# Autodesk Inventor assembly: WANYOIKE
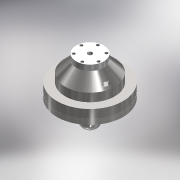
[picture p0: Inventor's stored thumbnail of the model, 180x180]
Saved by Autodesk Inventor 2021 (Build 250183000, 183)
## iProperties
Created: 2022-09-20
Part Number: WANYOIKE
Document SubType Name: Assembly
Designer: pc
Author: pc
## Documents named in this file (6)
- C:\Users\pc\Documents\injector\WANYOIKE.iam
- C:\Users\pc\Documents\injector\final injector body.ipt
- C:\Users\pc\Documents\injector\Orifice Plate.ipt
- C:\Users\pc\Documents\injector\Pintle tip vip.ipt
- C:\Users\pc\Documents\injector\pintle body.ipt
- C:\Users\pc\Documents\injector\faceplate.ipt
## Components (5 placed, 5 different names)
1. final injector body:1 — Mate:1, Rotational:1, Mate:2, Rotational:2, Mate:3, Rotational:4
2. Pintle tip vip:1 — Mate:3, Rotational:3, Mate:4
3. pintle body:1 — Mate:2, Rotational:2, Rotational:3
4. faceplate:1 — Mate:4, Rotational:4
5. Orifice Plate:1 — Mate:1, Rotational:1
## Relationships (8: Mate 4, RevoluteJoint 4)
- Mate:1: final injector body:1 ↔ Orifice Plate:1
- Rotational:1 [RevoluteJoint]: final injector body:1 ↔ Orifice Plate:1
- Mate:2: final injector body:1 ↔ pintle body:1
- Rotational:2 [RevoluteJoint]: final injector body:1 ↔ pintle body:1
- Mate:3: final injector body:1 ↔ Pintle tip vip:1
- Rotational:3 [RevoluteJoint]: Pintle tip vip:1 ↔ pintle body:1
- Mate:4: Pintle tip vip:1 ↔ faceplate:1
- Rotational:4 [RevoluteJoint]: final injector body:1 ↔ faceplate:1
